# Autodesk Inventor assembly: TestingPlatform_Assembly
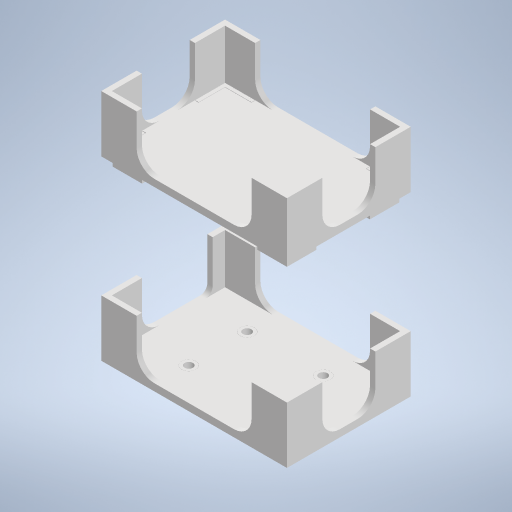
[picture p0: Inventor's stored thumbnail of the model, 512x512]
Saved by Autodesk Inventor 2024.2 (Build 282272000, 272)
## iProperties
Created: 2024-01-30
Part Number: TestingPlatform_Assembly
Document SubType Name: Assembly
Designer: ringl
Author: ringl
## Documents named in this file (5)
- C:\Users\ringl\OneDrive\Uni_PC_backup\Y4S2\EE579\Assignment\EE579-Skittles\CAD\TestingPlatform\TestingPlatform_Assembly.iam
- C:\Users\ringl\OneDrive\Uni_PC_backup\Y4S2\EE579\Assignment\EE579-Skittles\CAD\TestingPlatform\TestingPlatform_base01.ipt
- C:\Users\ringl\OneDrive\Uni_PC_backup\Y4S2\EE579\Assignment\EE579-Skittles\CAD\TestingPlatform\TestingPlatform_legs01.ipt
- C:\Users\ringl\OneDrive\Uni_PC_backup\Y4S2\EE579\Assignment\EE579-Skittles\CAD\TestingPlatform\TestingPlatform_standardStack01.ipt
- C:\Users\ringl\OneDrive\Uni_PC_backup\Y4S2\EE579\Assignment\EE579-Skittles\CAD\TestingPlatform\TestingPlatform_stackFeet01.ipt
## Components (10 placed, 4 different names)
1. TestingPlatform_base01:1 — Mate:1, Mate:2, Mate:3, Mate:4, Flush:1, Flush:2, Flush:3, Flush:4, Flush:8, Flush:9
2. TestingPlatform_legs01:1 — Mate:4, Flush:2
3. TestingPlatform_legs01:2 — Mate:1, Flush:1
4. TestingPlatform_legs01:3 — Mate:3, Flush:4
5. TestingPlatform_legs01:4 — Mate:2, Flush:3
6. TestingPlatform_standardStack01:1 — Mate:5, Mate:6, Mate:7, Mate:8, Mate:9, Flush:5, Mate:10, Mate:11, Flush:6, Mate:12, Mate:13, Flush:7, Flush:8, Flush:9
7. TestingPlatform_stackFeet01:1 — Mate:8, Mate:9, Flush:5
8. TestingPlatform_stackFeet01:2 — Mate:12, Mate:13, Flush:7
9. TestingPlatform_stackFeet01:3 — Mate:10, Mate:11, Flush:6
10. TestingPlatform_stackFeet01:4 — Mate:5, Mate:6, Mate:7
## Relationships (22: Mate 13, Flush 9)
- Mate:1: TestingPlatform_base01:1 ↔ TestingPlatform_legs01:2
- Mate:2: TestingPlatform_base01:1 ↔ TestingPlatform_legs01:4
- Mate:3: TestingPlatform_base01:1 ↔ TestingPlatform_legs01:3
- Mate:4: TestingPlatform_base01:1 ↔ TestingPlatform_legs01:1
- Flush:1: TestingPlatform_base01:1 ↔ TestingPlatform_legs01:2
- Flush:2: TestingPlatform_base01:1 ↔ TestingPlatform_legs01:1
- Flush:3: TestingPlatform_base01:1 ↔ TestingPlatform_legs01:4
- Flush:4: TestingPlatform_base01:1 ↔ TestingPlatform_legs01:3
- Mate:5: TestingPlatform_standardStack01:1 ↔ TestingPlatform_stackFeet01:4
- Mate:6: TestingPlatform_standardStack01:1 ↔ TestingPlatform_stackFeet01:4
- Mate:7: TestingPlatform_standardStack01:1 ↔ TestingPlatform_stackFeet01:4
- Mate:8: TestingPlatform_standardStack01:1 ↔ TestingPlatform_stackFeet01:1
- Mate:9: TestingPlatform_standardStack01:1 ↔ TestingPlatform_stackFeet01:1
- Flush:5: TestingPlatform_standardStack01:1 ↔ TestingPlatform_stackFeet01:1
- Mate:10: TestingPlatform_standardStack01:1 ↔ TestingPlatform_stackFeet01:3
- Mate:11: TestingPlatform_standardStack01:1 ↔ TestingPlatform_stackFeet01:3
- Flush:6: TestingPlatform_standardStack01:1 ↔ TestingPlatform_stackFeet01:3
- Mate:12: TestingPlatform_standardStack01:1 ↔ TestingPlatform_stackFeet01:2
- Mate:13: TestingPlatform_standardStack01:1 ↔ TestingPlatform_stackFeet01:2
- Flush:7: TestingPlatform_standardStack01:1 ↔ TestingPlatform_stackFeet01:2
- Flush:8: TestingPlatform_base01:1 ↔ TestingPlatform_standardStack01:1
- Flush:9: TestingPlatform_base01:1 ↔ TestingPlatform_standardStack01:1
